# Autodesk Inventor assembly: Assembly_cellphoneadapter
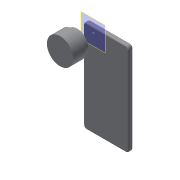
[picture p0: Inventor's stored thumbnail of the model, 180x180]
Saved by Autodesk Inventor 2019 (Build 230136000, 136)
## iProperties
Created: 2019-05-31
Part Number: Assembly_cellphoneadapter
Document SubType Name: Assembly
Designer: diederichbenedict
Author: diederichbenedict
## Documents named in this file (3)
- C:\Users\diederichbenedict\Dropbox\Dokumente\Promotion\PROJECTS\STORMoChip\INVENTOR\Nanoscopy-on-a-cheap\Assembly_cellphoneadapter.iam
- C:\Users\diederichbenedict\Dropbox\Dokumente\Promotion\PROJECTS\STORMoChip\INVENTOR\Nanoscopy-on-a-cheap\100.ipt
- C:\Users\diederichbenedict\Dropbox\Dokumente\Promotion\PROJECTS\STORMoChip\INVENTOR\Nanoscopy-on-a-cheap\100_Huawei_P9.ipt
## Components (2 placed, 2 different names)
1. 100:1 — Flush:1, Flush:2
2. 100_Huawei_P9:1 — Flush:1, Flush:2
## Relationships (2: Flush 2)
- Flush:1: 100:1 ↔ 100_Huawei_P9:1
- Flush:2 (24.8 mm): 100:1 ↔ 100_Huawei_P9:1
